# Autodesk Inventor assembly: UBG-Kamera mit Halter
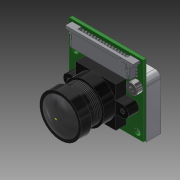
[picture p0: Inventor's stored thumbnail of the model, 180x180]
Saved by Autodesk Inventor 2019.1 (Build 231200000, 200)
## iProperties
Part Number: UBG-Kamera mit Halter
Material: Generisch
Document SubType Name: Assembly
Designer: rYan
Mass: 6.86612 g
Surface Area: 54.525 cm^2
Volume: 4.52999 cm^3
Density: 1.5157 g/cm^3
Author: rYan
## Documents named in this file (4)
- D:\TIGERsGIT\Hardware\mechanik\2019\Inventor\Elektronik\UBG-Kamera mit Halter.iam
- D:\TIGERsGIT\Hardware\mechanik\2019\Inventor\Elektronik\Kamerahalter Vorne.ipt
- D:\TIGERsGIT\Hardware\mechanik\2019\Inventor\Kaufteile\Waveshare Kamera 25x24\MG-Waveshare Kamera 25x24.iam
- D:\TIGERsGIT\Hardware\mechanik\2019\Inventor\Inhaltscenter\de-DE\ISO 4762(2)\ISO 4762 - M2 x 6ISO.ipt
## Components (4 placed, 3 different names)
1. Kamerahalter Vorne:1 — Fluchtend:1, Fluchtend:2, Fluchtend:3, Einfügen:1, Passend:1
2. MG-Waveshare Kamera 25x24:1 [sub-assembly] — Einfügen:1, Passend:1, Einfügen:2, Einfügen:3
3. ISO 4762 M2 x 6:1 — Einfügen:3
4. ISO 4762 M2 x 6:2 — Einfügen:2
## Relationships (7: Flush 3, Insert 3, Mate 1)
- Fluchtend:1 [Flush]: Kamerahalter Vorne:1
- Fluchtend:2 [Flush]: Kamerahalter Vorne:1
- Fluchtend:3 [Flush]: Kamerahalter Vorne:1
- Einfügen:1 [Insert]: Kamerahalter Vorne:1 ↔ MG-Waveshare Kamera 25x24:1
- Passend:1 [Mate]: Kamerahalter Vorne:1 ↔ MG-Waveshare Kamera 25x24:1
- Einfügen:2 [Insert]: MG-Waveshare Kamera 25x24:1 ↔ ISO 4762 M2 x 6:2
- Einfügen:3 [Insert]: MG-Waveshare Kamera 25x24:1 ↔ ISO 4762 M2 x 6:1
